# Autodesk Inventor assembly: SM_YA02
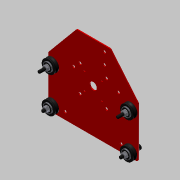
[picture p0: Inventor's stored thumbnail of the model, 180x180]
Saved by Autodesk Inventor 2012 SP1 (Build 160190100, 190)
## iProperties
Created: 2012-05-01
Part Number: SM_YA02
Document SubType Name: Assembly
Designer: ERF
Stock Number: SM_YA02
Mass: 349.48 g
Surface Area: 664.237 cm^2
Volume: 53.4389 cm^3
Density: 6.53981 g/cm^3
Author: ERF
Title: Y Axis Idle Mount Assembly
## Documents named in this file (7)
- C:\Users\eford\Documents\Projects\Shapoko_v1i\Workspaces\Workspace\Projects\USER FOLDER\Edward\Shapeoko_v1i\Assemblies\SM-YA02.iam
- C:\Users\eford\Documents\Projects\Shapoko_v1i\Workspaces\Workspace\Projects\USER FOLDER\Edward\Shapeoko_v1i\Parts\SM-S01.ipt
- C:\Users\eford\Documents\Projects\Shapoko_v1i\Workspaces\Workspace\Projects\USER FOLDER\Edward\Shapeoko_v1i\Parts\SM-H04.ipt
- C:\Users\eford\Documents\Projects\Shapoko_v1i\Workspaces\Workspace\Projects\USER FOLDER\Edward\Shapeoko_v1i\Parts\SM-H08.ipt
- C:\Users\eford\Documents\Projects\Shapoko_v1i\Workspaces\Workspace\Projects\USER FOLDER\Edward\Shapeoko_v1i\Parts\MSK01-04.ipt
- C:\Users\eford\Documents\Projects\Shapoko_v1i\Workspaces\Workspace\Projects\USER FOLDER\Edward\Shapeoko_v1i\Parts\SM-H03.ipt
- C:\Users\eford\Documents\Projects\Shapoko_v1i\Workspaces\Workspace\Projects\USER FOLDER\Edward\Shapeoko_v1i\Assemblies\MSK01-05A.iam
## Components (27 placed, 6 different names)
1. SM-S01:1 — Insert:27, Mate:3, Insert:29, Mate:5, Insert:33, Insert:34, Insert:35, Insert:36
2. SM-H08:1 — Insert:1
3. SM-H04:2 — Insert:23
4. SM-H08:2 — Insert:2
5. MSK01-05A:6 [sub-assembly] — Insert:43, Insert:44
6. SM-H04:3 — Insert:24
7. SM-H08:3 — Insert:3, Insert:7, Mate:1, Mate:2
8. MSK01-04:1 — Insert:7, Insert:27
9. SM-H04:4 — Insert:25
10. MSK01-05A:7 [sub-assembly] — Insert:37, Insert:38
11. MSK01-05A:8 [sub-assembly] — Insert:39, Insert:40
12. SM-H03:5 — Insert:3
13. SM-H03:6 — Insert:2, Insert:33
14. SM-H03:7 — Insert:1, Insert:35
15. SM-H03:8 — Insert:34, Insert:39
16. SM-H03:10 — Insert:24, Insert:38
17. SM-H03:11 — Insert:36, Insert:37
18. SM-H03:15 — Insert:25, Insert:44
19. SM-H03:17 — Insert:23, Insert:40
20. SM-H03:19 — Mate:1, Mate:2, Mate:3, Insert:43
21. SM-H08:4 — Insert:26, Mate:4
22. SM-H03:20 — Mate:4, Mate:5, Insert:41
23. MSK01-04:2 — Insert:28, Insert:29
24. MSK01-05A:9 [sub-assembly] — Insert:41, Insert:42
25. SM-H03:21 — Insert:32, Insert:42
26. SM-H04:5 — Insert:32
27. SM-H03:22 — Insert:26, Insert:28
## Relationships (29: Insert 24, Mate 5)
- Insert:1: SM-H08:1 ↔ SM-H03:7
- Insert:2: SM-H08:2 ↔ SM-H03:6
- Insert:3: SM-H08:3 ↔ SM-H03:5
- Insert:7: SM-H08:3 ↔ MSK01-04:1
- Mate:1: SM-H08:3 ↔ SM-H03:19
- Insert:23: SM-H04:2 ↔ SM-H03:17
- Insert:24: SM-H04:3 ↔ SM-H03:10
- Insert:25: SM-H04:4 ↔ SM-H03:15
- Insert:26: SM-H08:4 ↔ SM-H03:22
- Insert:27: SM-S01:1 ↔ MSK01-04:1
- Mate:2: SM-H08:3 ↔ SM-H03:19
- Mate:3: SM-S01:1 ↔ SM-H03:19
- Insert:28: MSK01-04:2 ↔ SM-H03:22
- Insert:29: SM-S01:1 ↔ MSK01-04:2
- Mate:4: SM-H08:4 ↔ SM-H03:20
- Mate:5: SM-S01:1 ↔ SM-H03:20
- Insert:32: SM-H03:21 ↔ SM-H04:5
- Insert:33: SM-S01:1 ↔ SM-H03:6
- Insert:34: SM-S01:1 ↔ SM-H03:8
- Insert:35: SM-S01:1 ↔ SM-H03:7
- Insert:36: SM-S01:1 ↔ SM-H03:11
- Insert:37: MSK01-05A:7 ↔ SM-H03:11
- Insert:38: MSK01-05A:7 ↔ SM-H03:10
- Insert:39: MSK01-05A:8 ↔ SM-H03:8
- Insert:40: MSK01-05A:8 ↔ SM-H03:17
- Insert:41: SM-H03:20 ↔ MSK01-05A:9
- Insert:42: MSK01-05A:9 ↔ SM-H03:21
- Insert:43: MSK01-05A:6 ↔ SM-H03:19
- Insert:44: MSK01-05A:6 ↔ SM-H03:15
